# Autodesk Inventor assembly: Claw Assembly
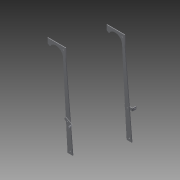
[picture p0: Inventor's stored thumbnail of the model, 180x180]
Saved by Autodesk Inventor 2013 (Build 170138000, 138)
## iProperties
Created: 2013-02-07
Part Number: Claw Assembly
Document SubType Name: Assembly
Designer: motoennies
Author: motoennies
## Documents named in this file (3)
- E:\Robotics\Climber\Claw Assembly.iam
- E:\Robotics\Climber\PassiveHooks2.ipt
- E:\Robotics\Climber\PistonFrontHinge.ipt
## Components (4 placed, 2 different names)
1. PassiveHooks2:1 — Mate:1, Mate:2
2. PassiveHooks2:2 — Mate:3, Mate:4
3. PistonFrontHinge:1 — Mate:1, Mate:2
4. PistonFrontHinge:2 — Mate:3, Mate:4
## Relationships (4: Mate 4)
- Mate:1: PassiveHooks2:1 ↔ PistonFrontHinge:1
- Mate:2: PassiveHooks2:1 ↔ PistonFrontHinge:1
- Mate:3: PassiveHooks2:2 ↔ PistonFrontHinge:2
- Mate:4: PassiveHooks2:2 ↔ PistonFrontHinge:2
